# Autodesk Inventor assembly: Arm
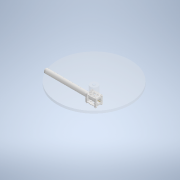
[picture p0: Inventor's stored thumbnail of the model, 180x180]
Saved by Autodesk Inventor 2022 (Build 260153000, 153)
## iProperties
Created: 2022-03-16
Part Number: Arm
Document SubType Name: Assembly
Designer: ARRF
Author: ARRF
## Documents named in this file (7)
- C:\Users\ARRF\Desktop\X500_prop\Arm\Arm.iam
- C:\Users\ARRF\Desktop\X500_prop\CAD\archive_ab8d35b\x500-kit\Frame Models\BAN-DJ.ipt
- C:\Users\ARRF\Desktop\X500_prop\CAD\archive_ab8d35b\x500-kit\Frame Models\GUAN-JIBI.ipt
- C:\Users\ARRF\Desktop\X500_prop\CAD\archive_ab8d35b\x500-kit\Frame Models\JIBI-JIA.ipt
- C:\Users\ARRF\Desktop\X500_prop\CAD\archive_ab8d35b\x500-kit\Frame Models\M3-30-PAN-DING.ipt
- C:\Users\ARRF\Desktop\X500_prop\CAD\archive_ab8d35b\x500-kit\Frame Models\ZSLM-M3-DING.ipt
- C:\Users\ARRF\Desktop\X500_prop\Arm\motor_with_prop.ipt
## Components (16 placed, 6 different names)
1. BAN-DJ:1 — Mate:1, Mate:2, Mate:3, Symmetry:1, Angle:4, Mate:12, Mate:13
2. BAN-DJ:2 — Mate:1, Mate:2, Mate:3, Symmetry:1, Flush:1, Angle:1, Angle:2, Angle:3, Mate:11, Mate:14, Mate:15, Mate:16
3. GUAN-JIBI:1 — Mate:6, Flush:1, Mate:7, Mate:8, Mate:9, Mate:10
4. JIBI-JIA:1 — Mate:7, Angle:1
5. JIBI-JIA:2 — Mate:8, Angle:2
6. JIBI-JIA:3 — Mate:10, Angle:4
7. JIBI-JIA:4 — Mate:9, Angle:3
8. motor_with_prop:1 — Mate:15, Mate:16
9. M3-30-PAN-DING:1 — Mate:11, Mate:14
10. ZSLM-M3-DING:1 — Mate:12, Mate:13
11. M3-30-PAN-DING:2
12. ZSLM-M3-DING:2
13. M3-30-PAN-DING:3
14. ZSLM-M3-DING:3
15. M3-30-PAN-DING:4
16. ZSLM-M3-DING:4
## Component patterns: (4 elements, first: M3-30-PAN-DING:1 + ZSLM-M3-DING:1)
## Relationships (22: Mate 16, Angle 4, Symmetry 1, Flush 1)
- Mate:1 (22.3 mm): BAN-DJ:1 ↔ BAN-DJ:2
- Mate:2: BAN-DJ:1 ↔ BAN-DJ:2
- Mate:3: BAN-DJ:1 ↔ BAN-DJ:2
- Symmetry:1: BAN-DJ:1 ↔ BAN-DJ:2
- Mate:4
- Mate:5
- Mate:6: GUAN-JIBI:1
- Flush:1: BAN-DJ:2 ↔ GUAN-JIBI:1
- Mate:7: GUAN-JIBI:1 ↔ JIBI-JIA:1
- Angle:1 (0 deg): BAN-DJ:2 ↔ JIBI-JIA:1
- Mate:8: GUAN-JIBI:1 ↔ JIBI-JIA:2
- Angle:2 (180 deg): BAN-DJ:2 ↔ JIBI-JIA:2
- Mate:9: GUAN-JIBI:1 ↔ JIBI-JIA:4
- Mate:10: GUAN-JIBI:1 ↔ JIBI-JIA:3
- Angle:3 (180 deg): BAN-DJ:2 ↔ JIBI-JIA:4
- Angle:4 (180 deg): BAN-DJ:1 ↔ JIBI-JIA:3
- Mate:11: BAN-DJ:2 ↔ M3-30-PAN-DING:1
- Mate:12: BAN-DJ:1 ↔ ZSLM-M3-DING:1
- Mate:13: BAN-DJ:1 ↔ ZSLM-M3-DING:1
- Mate:14: BAN-DJ:2 ↔ M3-30-PAN-DING:1
- Mate:15: BAN-DJ:2 ↔ motor_with_prop:1
- Mate:16: BAN-DJ:2 ↔ motor_with_prop:1
